# Autodesk Inventor assembly: Assembly3
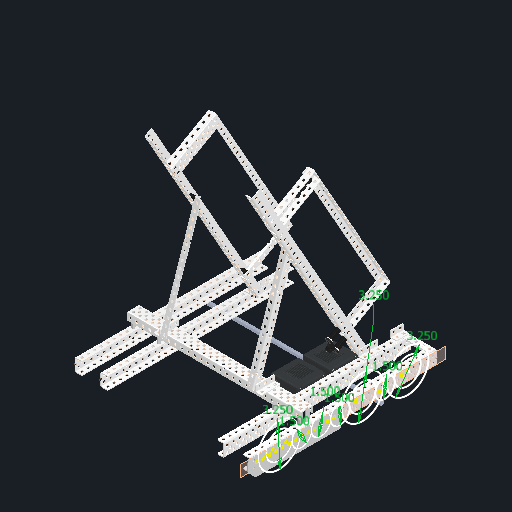
[picture p0: Inventor's stored thumbnail of the model, 512x512]
Saved by Autodesk Inventor 2025 (Build 290162010, 162A)
## iProperties
Created: 2025-10-28
Part Number: Assembly3
Document SubType Name: Assembly
Designer: jasper
Author: jasper
## iProperties of the stored document Standoff 1.00.ipt
Created: 2020-07-20
Part Number: Standoff .5
Material: VEX Aluminum Alloy 5052-H32
Document SubType Name: Modeling
Designer: yuany
Density: 2.68277 g/cm^3
Appearance: Default
Sending System: Autodesk Inventor 2026
Author: yuany
## Documents named in this file (25)
- C:\3284b-cad-2025\Assembly3.iam
- C:\3284b-cad-2025\Library\VEX-CAD-Inventor-1.4.2\Structure\C Channel\Aluminum 1x2x1\Alu C 1x2x1x29.ipt
- C:\3284b-cad-2025\Library\VEX-CAD-Inventor-1.4.2\Structure\C Channel\Aluminum 1x2x1\Alu C 1x2x1x27.ipt
- **C:\3284b-cad-2025\Assembly3.iam*LocalDocs*xAaaaaydaAaaaaaaaAaaaquvbXc*Standoff 1.00.ipt
- C:\3284b-cad-2025\Library\VEX-CAD-Inventor-1.4.2\Structure\Angle\Aluminum 1x1\Alu Angle 1x1x3.ipt
- C:\3284b-cad-2025\Library\VEX-CAD-Inventor-1.4.2\Structure\Angle\Aluminum 1x1\Alu Angle 1x1x17.ipt
- C:\3284b-cad-2025\Library\VEX-CAD-Inventor-1.4.2\Structure\C Channel\Aluminum 1x3x1 Half Thick Cut\Alu C Half Thick 1x3x1x34.ipt
- C:\3284b-cad-2025\Library\VEX-CAD-Inventor-1.4.2\Electronics\V5 Motor.ipt
- C:\3284b-cad-2025\Library\VEX-CAD-Inventor-1.4.2\Motion\Spacers\Spacer Nylon .375 OD\NSpacer .375 OD x .500.ipt
- C:\3284b-cad-2025\Library\VEX-CAD-Inventor-1.4.2\Motion\Spacers\Spacer Nylon .375 OD.ipt
- C:\3284b-cad-2025\Library\VEX-CAD-Inventor-1.4.2\Motion\Spacers\Spacer Nylon .375 OD\NSpacer .375 OD x .250.ipt
- C:\3284b-cad-2025\Library\VEX-CAD-Inventor-1.4.2\Motion\Spacers\Washer Teflon\TWasher .375 OD x .06250.ipt
- C:\3284b-cad-2025\Library\VEX-CAD-Inventor-1.4.2\Motion\Spacers\Washer Teflon.ipt
- C:\3284b-cad-2025\Library\VEX-CAD-Inventor-1.4.2\Motion\Shaft LS\LS Pillow Bearing Block.ipt
- C:\3284b-cad-2025\Library\VEX-CAD-Inventor-1.4.2\Structure\Angle\Aluminum 1x1\Alu Angle 1x1x8.ipt
- C:\3284b-cad-2025\Library\VEX-CAD-Inventor-1.4.2\Structure\C Channel\Aluminum 1x2x1\Alu C 1x2x1x8.ipt
- C:\3284b-cad-2025\Library\VEX-CAD-Inventor-1.4.2\Structure\Angle\Aluminum 1x1\Alu Angle 1x1x24.ipt
- C:\3284b-cad-2025\Library\VEX-CAD-Inventor-1.4.2\Motion\Shaft LS\Bearing Flat.ipt
- C:\3284b-cad-2025\Library\VEX-CAD-Inventor-1.4.2\Structure\Angle\Aluminum 1x1\Alu Angle 1x1x2.ipt
- C:\3284b-cad-2025\Library\VEX-CAD-Inventor-1.4.2\Motion\Shaft HS\Shaft HS\Shaft HS 13.5 in.ipt
- C:\3284b-cad-2025\Library\VEX-CAD-Inventor-1.4.2\Motion\Shaft HS\Shaft HS.ipt
- C:\3284b-cad-2025\Part1.ipt
- C:\3284b-cad-2025\Part2.ipt
- C:\3284b-cad-2025\Library\VEX-CAD-Inventor-1.4.2\Structure\C Channel\Aluminum 1x3x1 Half Thick Cut\Alu C Half Thick 1x3x1x5.ipt
- C:\3284b-cad-2025\Library\VEX-CAD-Inventor-1.4.2\Structure\Standoff\Standoff 1.00.ipt
## Components (53 placed, 20 different names)
1. Alu C 1x2x1x29:1 — Insert:7, Insert:8, Flush:2, Mate:1, Flush:3, Flush:4, Insert:74
2. Alu C 1x2x1x29:2 — Insert:5, Insert:6, Insert:24, Insert:25, Insert:30, Insert:31, Insert:32, Insert:33, Insert:53, Insert:73
3. Alu C 1x2x1x29:3 — Insert:3, Insert:4, Insert:26, Insert:27
4. Alu C 1x2x1x29:4 — Insert:1, Insert:2
5. Alu C 1x2x1x27:1 — Insert:9, Insert:11, Insert:12, Insert:13, Insert:14, Insert:15, Insert:16, Insert:17, Insert:18, Insert:19, Insert:20, Insert:21
6. Standoff 1.00:1 — Insert:1, Insert:11
7. Standoff 1.00:2 — Insert:2, Insert:9
8. Standoff 1.00:3 — Insert:4, Insert:13
9. Standoff 1.00:4 — Insert:3, Insert:12
10. Standoff 1.00:5 — Insert:5, Insert:16
11. Standoff 1.00:6 — Insert:6, Insert:17
12. Standoff 1.00:7 — Insert:7, Insert:15
13. Standoff 1.00:8 — Insert:8, Insert:14
14. Alu Angle 1x1x3:1 — Insert:18, Insert:19, Insert:59, Insert:63
15. Alu Angle 1x1x3:2 — Insert:20, Insert:21, Insert:22
16. Alu Angle 1x1x17:1 — Insert:22, Insert:29, Insert:62, Insert:64
17. Alu Angle 1x1x3:3 — Insert:24, Insert:25, Insert:57
18. Alu Angle 1x1x3:4 — Insert:26, Insert:27, Insert:58
19. Alu C Half Thick 1x3x1x34:1 — Insert:29, Insert:40, Insert:41, Insert:42, Insert:44, Insert:45, Insert:57
20. V5 Motor:1 — Insert:30, Insert:31
21. V5 Motor:2 — Insert:32, Insert:33
22. NSpacer .375 OD x .500:1 — Insert:35, Insert:41
23. NSpacer .375 OD x .250:2 — Insert:34, Insert:35
24. TWasher .375 OD x .06250:1 — Insert:34, Insert:39
25. LS Pillow Bearing Block:1 — Insert:38, Insert:39
26. NSpacer .375 OD x .500:3 — Insert:40
27. NSpacer .375 OD x .250:4
28. TWasher .375 OD x .06250:2 — Insert:38
29. NSpacer .375 OD x .500:5 — Insert:42, Insert:43
30. Alu Angle 1x1x8:1 — Insert:43, Insert:50
31. Alu C 1x2x1x8:1 — Insert:46, Insert:47, Insert:48, Insert:49, Insert:51, Insert:52
32. NSpacer .375 OD x .500:6 — Insert:44, Insert:47
33. NSpacer .375 OD x .500:7 — Insert:45, Insert:46
34. Alu Angle 1x1x24:1 — Insert:48, Insert:49, Insert:50
35. Bearing Flat:1 — Insert:51, Insert:52
36. Alu Angle 1x1x2:1 — Insert:55
37. TWasher .375 OD x .06250:3 — Insert:53, Insert:55
38. Shaft HS 13.5 in:1 — Flush:2, Mate:1
39. Part1:1 — Flush:3
40. Part2:1 — Flush:4
41. Alu C Half Thick 1x3x1x34:2 — Insert:58, Insert:60, Insert:65, Insert:72
42. Alu Angle 1x1x17:2 — Insert:59, Insert:61
43. NSpacer .375 OD x .500:8 — Insert:60, Insert:61
44. NSpacer .375 OD x .500:9 — Insert:62
45. TWasher .375 OD x .06250:5 — Insert:63
46. TWasher .375 OD x .06250:6 — Insert:64
47. Alu Angle 1x1x8:2 — Insert:66, Insert:67
48. NSpacer .375 OD x .500:10 — Insert:65, Insert:66
49. Alu Angle 1x1x24:2 — Insert:67, Insert:68, Insert:69
50. Alu C 1x2x1x8:2 — Insert:68, Insert:69, Insert:70, Insert:71
51. NSpacer .375 OD x .500:11 — Insert:70
52. NSpacer .375 OD x .500:12 — Insert:71, Insert:72
53. Alu C Half Thick 1x3x1x5:1 — Insert:73, Insert:74
## Relationships (73: Insert 69, Flush 3, Mate 1)
- Insert:1: Alu C 1x2x1x29:4 ↔ Standoff 1.00:1
- Insert:2: Alu C 1x2x1x29:4 ↔ Standoff 1.00:2
- Insert:3: Alu C 1x2x1x29:3 ↔ Standoff 1.00:4
- Insert:4: Alu C 1x2x1x29:3 ↔ Standoff 1.00:3
- Insert:5: Alu C 1x2x1x29:2 ↔ Standoff 1.00:5
- Insert:6: Alu C 1x2x1x29:2 ↔ Standoff 1.00:6
- Insert:7: Alu C 1x2x1x29:1 ↔ Standoff 1.00:7
- Insert:8: Alu C 1x2x1x29:1 ↔ Standoff 1.00:8
- Insert:9: Alu C 1x2x1x27:1 ↔ Standoff 1.00:2
- Insert:11: Alu C 1x2x1x27:1 ↔ Standoff 1.00:1
- Insert:12: Alu C 1x2x1x27:1 ↔ Standoff 1.00:4
- Insert:13: Alu C 1x2x1x27:1 ↔ Standoff 1.00:3
- Insert:14: Alu C 1x2x1x27:1 ↔ Standoff 1.00:8
- Insert:15: Alu C 1x2x1x27:1 ↔ Standoff 1.00:7
- Insert:16: Alu C 1x2x1x27:1 ↔ Standoff 1.00:5
- Insert:17: Alu C 1x2x1x27:1 ↔ Standoff 1.00:6
- Insert:18 (1.5875 mm): Alu C 1x2x1x27:1 ↔ Alu Angle 1x1x3:1
- Insert:19 (1.5875 mm): Alu C 1x2x1x27:1 ↔ Alu Angle 1x1x3:1
- Insert:20 (1.5875 mm): Alu C 1x2x1x27:1 ↔ Alu Angle 1x1x3:2
- Insert:21 (1.5875 mm): Alu C 1x2x1x27:1 ↔ Alu Angle 1x1x3:2
- Insert:22 (1.5875 mm): Alu Angle 1x1x3:2 ↔ Alu Angle 1x1x17:1
- Insert:24: Alu C 1x2x1x29:2 ↔ Alu Angle 1x1x3:3
- Insert:25: Alu C 1x2x1x29:2 ↔ Alu Angle 1x1x3:3
- Insert:26: Alu C 1x2x1x29:3 ↔ Alu Angle 1x1x3:4
- Insert:27: Alu C 1x2x1x29:3 ↔ Alu Angle 1x1x3:4
- Insert:29 (12.7 mm): Alu Angle 1x1x17:1 ↔ Alu C Half Thick 1x3x1x34:1
- Insert:30: Alu C 1x2x1x29:2 ↔ V5 Motor:1
- Insert:31: Alu C 1x2x1x29:2 ↔ V5 Motor:1
- Insert:32: Alu C 1x2x1x29:2 ↔ V5 Motor:2
- Insert:33: Alu C 1x2x1x29:2 ↔ V5 Motor:2
- Insert:34: NSpacer .375 OD x .250:2 ↔ TWasher .375 OD x .06250:1
- Insert:35: NSpacer .375 OD x .500:1 ↔ NSpacer .375 OD x .250:2
- [Insert]: NSpacer .375 OD x .250:4 ↔ TWasher .375 OD x .06250:2
- [Insert]: NSpacer .375 OD x .500:3 ↔ NSpacer .375 OD x .250:4
- Insert:38: LS Pillow Bearing Block:1 ↔ TWasher .375 OD x .06250:2
- Insert:39: TWasher .375 OD x .06250:1 ↔ LS Pillow Bearing Block:1
- Insert:40: Alu C Half Thick 1x3x1x34:1 ↔ NSpacer .375 OD x .500:3
- Insert:41: Alu C Half Thick 1x3x1x34:1 ↔ NSpacer .375 OD x .500:1
- Insert:42: Alu C Half Thick 1x3x1x34:1 ↔ NSpacer .375 OD x .500:5
- Insert:43: NSpacer .375 OD x .500:5 ↔ Alu Angle 1x1x8:1
- Insert:44: Alu C Half Thick 1x3x1x34:1 ↔ NSpacer .375 OD x .500:6
- Insert:45: Alu C Half Thick 1x3x1x34:1 ↔ NSpacer .375 OD x .500:7
- Insert:46: Alu C 1x2x1x8:1 ↔ NSpacer .375 OD x .500:7
- Insert:47: Alu C 1x2x1x8:1 ↔ NSpacer .375 OD x .500:6
- Insert:48: Alu C 1x2x1x8:1 ↔ Alu Angle 1x1x24:1
- Insert:49: Alu C 1x2x1x8:1 ↔ Alu Angle 1x1x24:1
- Insert:50: Alu Angle 1x1x8:1 ↔ Alu Angle 1x1x24:1
- Insert:51: Alu C 1x2x1x8:1 ↔ Bearing Flat:1
- Insert:52: Alu C 1x2x1x8:1 ↔ Bearing Flat:1
- Insert:53: Alu C 1x2x1x29:2 ↔ TWasher .375 OD x .06250:3
- Insert:55: Alu Angle 1x1x2:1 ↔ TWasher .375 OD x .06250:3
- Flush:2: Alu C 1x2x1x29:1 ↔ Shaft HS 13.5 in:1
- Mate:1 (7.9375 mm): Alu C 1x2x1x29:1 ↔ Shaft HS 13.5 in:1
- Flush:3: Alu C 1x2x1x29:1 ↔ Part1:1
- Insert:57: Alu Angle 1x1x3:3 ↔ Alu C Half Thick 1x3x1x34:1
- Flush:4: Alu C 1x2x1x29:1 ↔ Part2:1
- Insert:58: Alu Angle 1x1x3:4 ↔ Alu C Half Thick 1x3x1x34:2
- Insert:59 (1.5875 mm): Alu Angle 1x1x3:1 ↔ Alu Angle 1x1x17:2
- Insert:60: Alu C Half Thick 1x3x1x34:2 ↔ NSpacer .375 OD x .500:8
- Insert:61: Alu Angle 1x1x17:2 ↔ NSpacer .375 OD x .500:8
- Insert:62: Alu Angle 1x1x17:1 ↔ NSpacer .375 OD x .500:9
- Insert:63: Alu Angle 1x1x3:1 ↔ TWasher .375 OD x .06250:5
- Insert:64: Alu Angle 1x1x17:1 ↔ TWasher .375 OD x .06250:6
- Insert:65: Alu C Half Thick 1x3x1x34:2 ↔ NSpacer .375 OD x .500:10
- Insert:66: Alu Angle 1x1x8:2 ↔ NSpacer .375 OD x .500:10
- Insert:67: Alu Angle 1x1x8:2 ↔ Alu Angle 1x1x24:2
- Insert:68: Alu Angle 1x1x24:2 ↔ Alu C 1x2x1x8:2
- Insert:69: Alu Angle 1x1x24:2 ↔ Alu C 1x2x1x8:2
- Insert:70: Alu C 1x2x1x8:2 ↔ NSpacer .375 OD x .500:11
- Insert:71: Alu C 1x2x1x8:2 ↔ NSpacer .375 OD x .500:12
- Insert:72: Alu C Half Thick 1x3x1x34:2 ↔ NSpacer .375 OD x .500:12
- Insert:73: Alu C 1x2x1x29:2 ↔ Alu C Half Thick 1x3x1x5:1
- Insert:74: Alu C 1x2x1x29:1 ↔ Alu C Half Thick 1x3x1x5:1
## Named parameters: d59_d57 = 0 mm, d60_d58 = 0 mm
